# Autodesk Inventor assembly: Pneumatic Wheel
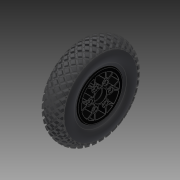
[picture p0: Inventor's stored thumbnail of the model, 180x180]
Saved by Autodesk Inventor 2014 SP1 (Build 180222100, 222)
## iProperties
Created: 2013-01-29
Part Number: Pneumatic Wheel
Document SubType Name: Assembly
Designer: actoennies
Mass: 512.559 g
Surface Area: 2399.32 cm^2
Volume: 453.254 cm^3
Density: 1.13084 g/cm^3
Translation Standard: STEP AP214IS
FileName: Pneumatic Wheel.STEP
PreProcessor: SolidWorks 2010
PostProcessor: Build: 138, Release: 2013 RTM - Date: Thu 03/01/2012
Sent Units: inch
Uncertainty: 1e-05
Author: actoennies
## Documents named in this file (4)
- C:\Users\Moses\Documents\Inventor\Rebuilds\Rebuild Sally\Pneumatic Wheel.iam
- C:\Users\Moses\Documents\Inventor\Rebuilds\Rebuild Sally\Tire.ipt
- C:\Users\Moses\Documents\Inventor\Rebuilds\Rebuild Sally\Valve.ipt
- C:\Users\Moses\Documents\Inventor\Rebuilds\Rebuild Sally\Pneumatic Hub.iam
## Components (3 placed, 3 different names)
1. Tire:1 — Mate:2
2. Valve:1 — Mate:1
3. Pneumatic Hub:1 [sub-assembly] — Mate:1, Mate:2
## Relationships (2: Mate 2)
- Mate:1: Valve:1 ↔ Pneumatic Hub:1
- Mate:2: Tire:1 ↔ Pneumatic Hub:1
